(part 1 of 2)
# Autodesk Inventor assembly: Почти готово_CPY
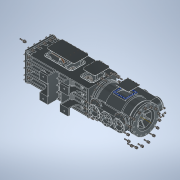
[picture p0: Inventor's stored thumbnail of the model, 180x180]
Saved by Autodesk Inventor 2021 (Build 250183000, 183)
## iProperties
Created: 2020-12-08
Part Number: Почти готово_CPY
Document SubType Name: Assembly
Designer: Тимоха
Author: Тимоха
## Documents named in this file (76)
- C:\Users\Тимоха\Desktop\КР Компрессор\compressor\Почти готово_CPY.iam
- C:\Users\Тимоха\Desktop\КР Компрессор\compressor\Фонарь_CPY.ipt
- C:\Users\Тимоха\Desktop\КР Компрессор\compressor\Башмак_CPY.ipt
- C:\Users\Тимоха\Desktop\КР Компрессор\compressor\Втулка палец шатун_CPY.ipt
- C:\Users\Тимоха\Desktop\КР Компрессор\compressor\Втулка под палец_CPY.ipt
- C:\Users\Тимоха\Desktop\КР Компрессор\compressor\Гайка шток_CPY.ipt
- C:\Users\Тимоха\Desktop\КР Компрессор\compressor\Крейцкопф_CPY.ipt
- C:\Users\Тимоха\Desktop\КР Компрессор\compressor\Палец_CPY.ipt
- C:\Users\Тимоха\Desktop\КР Компрессор\compressor\Стопорное кольцо_CPY.ipt
- C:\Users\Тимоха\Desktop\КР Компрессор\compressor\Верхняя часть поршня_CPY.ipt
- C:\Users\Тимоха\Desktop\КР Компрессор\compressor\Втулка_CPY.ipt
- C:\Users\Тимоха\Desktop\КР Компрессор\compressor\Гайка шток-поршень_CPY.ipt
- C:\Users\Тимоха\Desktop\КР Компрессор\compressor\Кольцо поршень-шток верх_CPY.ipt
- C:\Users\Тимоха\Desktop\КР Компрессор\compressor\Кольцо поршень-шток низ_CPY.ipt
- C:\Users\Тимоха\Desktop\КР Компрессор\compressor\Кольцо поршня_CPY.ipt
- C:\Users\Тимоха\Desktop\КР Компрессор\compressor\Кольцо сальника_CPY.ipt
- C:\Users\Тимоха\Desktop\КР Компрессор\compressor\Корпус дросселя_CPY.ipt
- C:\Users\Тимоха\Desktop\КР Компрессор\compressor\Корпус сальника_CPY.ipt
- C:\Users\Тимоха\Desktop\КР Компрессор\compressor\Крышка стакана_CPY.ipt
- C:\Users\Тимоха\Desktop\КР Компрессор\compressor\Крышка цилиндра 1_CPY.ipt
- C:\Users\Тимоха\Desktop\КР Компрессор\compressor\Крышка цилиндра 2_CPY.ipt
- C:\Users\Тимоха\Desktop\КР Компрессор\compressor\Нижняя часть поршня_CPY.ipt
- C:\Users\Тимоха\Desktop\КР Компрессор\compressor\Опорное кольцо_CPY.ipt
- C:\Users\Тимоха\Desktop\КР Компрессор\compressor\Пружина дросселя_CPY.ipt
- C:\Users\Тимоха\Desktop\КР Компрессор\compressor\Пружина сальника_CPY.ipt
- C:\Users\Тимоха\Desktop\КР Компрессор\compressor\Цилиндр2_CPY.ipt
- C:\Users\Тимоха\Desktop\КР Компрессор\compressor\Клапан1_CPY.iam
- C:\Users\Тимоха\Desktop\КР Компрессор\compressor\Прокладка клапана_CPY.ipt
- C:\Users\Тимоха\Desktop\КР Компрессор\compressor\Стакан1_CPY.ipt
- C:\Users\Тимоха\Desktop\КР Компрессор\compressor\Дроссельное кольцо_CPY.ipt
- C:\Users\Тимоха\Desktop\КР Компрессор\compressor\Уплотнительное кольцо_CPY.ipt
- C:\Users\Тимоха\Desktop\КР Компрессор\compressor\Уплотнение фонарь_CPY.ipt
- C:\Users\Тимоха\Desktop\КР Компрессор\compressor\Крышка сальников_CPY.ipt
- C:\Users\Тимоха\Desktop\КР Компрессор\compressor\Корпус маслосъемника_CPY.ipt
- C:\Users\Тимоха\Desktop\КР Компрессор\compressor\Корпус сальника перегородка 1_CPY.ipt
- C:\Users\Тимоха\Desktop\КР Компрессор\compressor\Крышка перегородки11_CPY.ipt
- C:\Users\Тимоха\Desktop\КР Компрессор\compressor\Крышка перегородки12_CPY.ipt
- C:\Users\Тимоха\Desktop\КР Компрессор\compressor\Крышка перегородки21_CPY.ipt
- C:\Users\Тимоха\Desktop\КР Компрессор\compressor\Крышка перегородки22_CPY.ipt
- C:\Users\Тимоха\Desktop\КР Компрессор\compressor\Маслосъемная пружина_CPY.ipt
- C:\Users\Тимоха\Desktop\КР Компрессор\compressor\Маслосъемное кольцо_CPY.ipt
- C:\Users\Тимоха\Desktop\КР Компрессор\compressor\Придав перегородки1_CPY.ipt
- C:\Users\Тимоха\Desktop\КР Компрессор\compressor\Фланецгайка_CPY.ipt
- C:\Users\Тимоха\Desktop\КР Компрессор\compressor\Шток_CPY.ipt
- C:\Users\Тимоха\Desktop\КР Компрессор\compressor\Прокладка крейцкопф_CPY.ipt
- C:\Users\Тимоха\Documents\Inventor\Content Center Files\R2021\ru-RU\Stud GOST 22038-76\Шпилька M24-6g×70 ГОСТ 22038-76.ipt
- C:\Users\Тимоха\Documents\Inventor\Content Center Files\R2021\ru-RU\Nut GOST 15524-70\Гайка M24-6H ГОСТ 15524-70.ipt
- C:\Users\Тимоха\Documents\Inventor\Content Center Files\R2021\ru-RU\GOST 11371-78  A\Шайба 24 ГОСТ 11371-78.ipt
- C:\Users\Тимоха\Documents\Inventor\Content Center Files\R2021\ru-RU\GOST 15521-70\Гайка M20-6H ГОСТ 15521-70.ipt
- C:\Users\Тимоха\Documents\Inventor\Content Center Files\R2021\ru-RU\Stud GOST 22034-76\Шпилька M20-6g×50 ГОСТ 22034-76.ipt
- C:\Users\Тимоха\Documents\Inventor\Content Center Files\R2021\ru-RU\GOST 10450-78\Шайба 19 ГОСТ 10450-78.ipt
- C:\Users\Тимоха\Documents\Inventor\Content Center Files\R2021\ru-RU\Stud GOST 22038-76\Шпилька M20-6g×85 ГОСТ 22038-76.ipt
- C:\Users\Тимоха\Documents\Inventor\Content Center Files\R2021\ru-RU\GOST 10450-78\Шайба 21 ГОСТ 10450-78.ipt
- C:\Users\Тимоха\Documents\Inventor\Content Center Files\R2021\ru-RU\Nut GOST 15524-70\Гайка M20-6H ГОСТ 15524-70.ipt
- C:\Users\Тимоха\Documents\Inventor\Content Center Files\R2021\ru-RU\GOST 11738-84\Винт M10-6gx35 ГОСТ 11738-84.ipt
- C:\Users\Тимоха\Documents\Inventor\Content Center Files\R2021\ru-RU\GOST 11371-78  A\Шайба 12 ГОСТ 11371-78.ipt
- C:\Users\Тимоха\Documents\Inventor\Content Center Files\R2021\ru-RU\GOST 11738-84\Винт M10-6gx30 ГОСТ 11738-84.ipt
- C:\Users\Тимоха\Documents\Inventor\Content Center Files\R2021\ru-RU\GOST 11738-84\Винт M10-6gx25 ГОСТ 11738-84.ipt
- C:\Users\Тимоха\Documents\Inventor\Content Center Files\R2021\ru-RU\Stud GOST 22038-76\Шпилька M24-6g×80 ГОСТ 22038-76.ipt
- C:\Users\Тимоха\Documents\Inventor\Content Center Files\R2021\ru-RU\GOST 11371-78  A\Шайба 27 ГОСТ 11371-78.ipt
- C:\Users\Тимоха\Desktop\КР Компрессор\compressor\Крышка стакана_MIR_CPY.ipt
- C:\Users\Тимоха\Desktop\КР Компрессор\compressor\Деталь5_CPY.ipt
- C:\Users\Тимоха\Desktop\КР Компрессор\compressor\Деталь6_CPY.ipt
- C:\Users\Тимоха\Documents\Inventor\Content Center Files\R2021\ru-RU\GOST 11371-78  A\Шайба 22 ГОСТ 11371-78.ipt
- C:\Users\Тимоха\Documents\Inventor\Content Center Files\R2021\ru-RU\Bolt GOST R 50274-92\Болт M8-6g×16-F ГОСТ Р 50274-92.ipt
- C:\Users\Тимоха\Desktop\КР Компрессор\compressor\Прокладка крышки фонаря 1_CPY.ipt
- C:\Users\Тимоха\Desktop\КР Компрессор\compressor\Прокладка крышки фонаря 2_CPY.ipt
- C:\Users\Тимоха\Desktop\КР Компрессор\compressor\Маслоотражательное кольцо_CPY.ipt
- C:\Users\Тимоха\Desktop\КР Компрессор\compressor\Прокладка крышки фонаря 1_CPY_MIR.ipt
- C:\Users\Тимоха\Desktop\КР Компрессор\compressor\Прокладка крышки фонаря 2_CPY_MIR.ipt
- C:\Users\Тимоха\Desktop\КР Компрессор\compressor\Крышка фонаря 1.ipt
- C:\Users\Тимоха\Desktop\КР Компрессор\compressor\Крышка фонаря 2.ipt
- C:\Users\Тимоха\Desktop\КР Компрессор\compressor\Крышка фонаря 1_MIR1.ipt
- C:\Users\Тимоха\Desktop\КР Компрессор\compressor\Крышка фонаря 2_MIR1.ipt
- C:\Users\Тимоха\Desktop\КР Компрессор\compressor\Деталь6_CPY_MIR.ipt
- C:\Users\Тимоха\Desktop\КР Компрессор\compressor\Деталь5_CPY_MIR.ipt
## Components (627 placed, 75 different names)
1. Фонарь_CPY:1 — Заподлицо:5, Заподлицо:4, Заподлицо:7, Заподлицо:6, Цилиндрический:2, Жесткий:70, Жесткий:69, Жесткий:94, Жесткий:98, Жесткий:97, Жесткий:106, Жесткий:127, Жесткий:163, Жесткий:165, Жесткий:166, Жесткий:164, Жесткий:171, Жесткий:173, Жесткий:174, Жесткий:172, Жесткий:169, Жесткий:167, Жесткий:170, Жесткий:168, Жесткий:192, Жесткий:197, Жесткий:191, Жесткий:196, Жесткий:194, Жесткий:193, Жесткий:195, Заподлицо:9, Заподлицо:10, Заподлицо:11, Заподлицо:12
2. Башмак_CPY:1 — Цилиндрический:2, Жесткий:4
3. Втулка палец шатун_CPY:1 — Жесткий:3
4. Втулка под палец_CPY:1 — Жесткий:1, С поворотом:1
5. Гайка шток_CPY:1 — Жесткий:110
6. Крейцкопф_CPY:1 — Жесткий:4, Жесткий:1, Жесткий:2, Жесткий:5, Жесткий:206, Жесткий:208, Жесткий:209
7. Втулка под палец_CPY:2 — Жесткий:3, Жесткий:2
8. Башмак_CPY:2 — Жесткий:5
9. Палец_CPY:1 — С поворотом:1, Жесткий:7, Жесткий:6
10. Стопорное кольцо_CPY:1 — Жесткий:7
11. Стопорное кольцо_CPY:2 — Жесткий:6
12. Верхняя часть поршня_CPY:1 — Совмещение:1, Жесткий:13, Жесткий:9, Жесткий:8, Жесткий:20
13. Втулка_CPY:1 — Жесткий:16, Жесткий:15, Цилиндрический:1
14. Гайка шток-поршень_CPY:1 — Жесткий:14, Жесткий:107
15. Кольцо поршень-шток верх_CPY:1 — Жесткий:14, Жесткий:13
16. Кольцо поршень-шток низ_CPY:1 — Жесткий:12
17. Кольцо поршня_CPY:1 — Жесткий:9
18. Кольцо сальника_CPY:1 — Жесткий:27, Жесткий:31, Жесткий:30
19. Корпус дросселя_CPY:1 — С поворотом:3, Жесткий:26, Жесткий:62
20. Корпус сальника_CPY:1 — С поворотом:3, Жесткий:32, Жесткий:57
21. Крышка стакана_CPY:1 — Жесткий:23
22. Крышка цилиндра 1_CPY:1 — Совмещение:1, Жесткий:16, Жесткий:112
23. Крышка цилиндра 2_CPY:1 — Жесткий:70, Жесткий:79, Жесткий:61, Жесткий:78, Жесткий:125
24. Нижняя часть поршня_CPY:1 — Жесткий:12, Жесткий:8, Жесткий:21, Жесткий:11, Жесткий:10
25. Опорное кольцо_CPY:1 — Жесткий:21
26. Пружина дросселя_CPY:1 — Жесткий:25
27. Пружина сальника_CPY:1 — Жесткий:27
28. Цилиндр2_CPY:1 — Заподлицо:2, Жесткий:79, Жесткий:23, Жесткий:15, Жесткий:80, Жесткий:18, Жесткий:81, Жесткий:111, Жесткий:116, Жесткий:115, Жесткий:117, Жесткий:118, Жесткий:119, Жесткий:122, Жесткий:461
29. Кольцо поршня_CPY:2 — Жесткий:11
30. Кольцо поршня_CPY:3 — Цилиндрический:1, Жесткий:10
31. Клапан1_CPY:1 [sub-assembly] — Жесткий:80
32. Прокладка клапана_CPY:1 — Жесткий:18
33. Стакан1_CPY:1 — Жесткий:81
34. Опорное кольцо_CPY:2 — Жесткий:20
35. Дроссельное кольцо_CPY:1 — Жесткий:26, Жесткий:25
36. Кольцо сальника_CPY:2 — Жесткий:32, Жесткий:31, Жесткий:28
37. Пружина сальника_CPY:2 — Жесткий:28
38. Кольцо сальника_CPY:3 — Жесткий:30, Жесткий:29
39. Пружина сальника_CPY:3 — Жесткий:29
40. Кольцо сальника_CPY:4 — Жесткий:33, Жесткий:37, Жесткий:36
41. Корпус сальника_CPY:2 — Жесткий:57, Жесткий:38, Жесткий:58
42. Пружина сальника_CPY:4 — Жесткий:33
43. Кольцо сальника_CPY:5 — Жесткий:38, Жесткий:37, Жесткий:34
44. Пружина сальника_CPY:5 — Жесткий:34
45. Кольцо сальника_CPY:6 — Жесткий:36, Жесткий:35
46. Пружина сальника_CPY:6 — Жесткий:35
47. Кольцо сальника_CPY:7 — Жесткий:39, Жесткий:43, Жесткий:42
48. Корпус сальника_CPY:3 — Жесткий:58, Жесткий:44, Жесткий:59
49. Пружина сальника_CPY:7 — Жесткий:39
50. Кольцо сальника_CPY:8 — Жесткий:44, Жесткий:43, Жесткий:40
51. Пружина сальника_CPY:8 — Жесткий:40
52. Кольцо сальника_CPY:9 — Жесткий:42, Жесткий:41
53. Пружина сальника_CPY:9 — Жесткий:41
54. Кольцо сальника_CPY:10 — Жесткий:45, Жесткий:49, Жесткий:48
55. Корпус сальника_CPY:4 — Жесткий:59, Жесткий:50, Жесткий:60
56. Пружина сальника_CPY:10 — Жесткий:45
57. Кольцо сальника_CPY:11 — Жесткий:50, Жесткий:49, Жесткий:46
58. Пружина сальника_CPY:11 — Жесткий:46
59. Кольцо сальника_CPY:12 — Жесткий:48, Жесткий:47
60. Пружина сальника_CPY:12 — Жесткий:47
61. Кольцо сальника_CPY:13 — Жесткий:51, Жесткий:55, Жесткий:54
62. Корпус сальника_CPY:5 — Жесткий:60, Жесткий:56, Жесткий:77
63. Пружина сальника_CPY:13 — Жесткий:51
64. Кольцо сальника_CPY:14 — Жесткий:56, Жесткий:55, Жесткий:52
65. Пружина сальника_CPY:14 — Жесткий:52
66. Кольцо сальника_CPY:15 — Жесткий:54, Жесткий:53
67. Пружина сальника_CPY:15 — Жесткий:53
68. Уплотнительное кольцо_CPY:1 — Жесткий:62, Жесткий:61
69. Кольцо сальника_CPY:16 — Жесткий:63, Жесткий:67, Жесткий:66
70. Пружина сальника_CPY:16 — Жесткий:63
71. Кольцо сальника_CPY:17 — Жесткий:67, Жесткий:64, Жесткий:103
72. Пружина сальника_CPY:17 — Жесткий:64
73. Кольцо сальника_CPY:18 — Жесткий:66, Жесткий:65
74. Пружина сальника_CPY:18 — Жесткий:65
75. Уплотнение фонарь_CPY:1 — Жесткий:69
76. Кольцо сальника_CPY:19 — Жесткий:71, Жесткий:75, Жесткий:74
77. Корпус сальника_CPY:6 — Жесткий:77, Жесткий:76
78. Пружина сальника_CPY:19 — Жесткий:71
79. Кольцо сальника_CPY:20 — Жесткий:76, Жесткий:75, Жесткий:72
80. Пружина сальника_CPY:20 — Жесткий:72
81. Кольцо сальника_CPY:21 — Жесткий:74, Жесткий:73
82. Пружина сальника_CPY:21 — Жесткий:73
83. Крышка сальников_CPY:1 — Жесткий:78
84. Корпус маслосъемника_CPY:1 — Жесткий:104, Жесткий:102
85. Корпус сальника перегородка 1_CPY:1 — Жесткий:95, Жесткий:96, Жесткий:87, Жесткий:93
86. Крышка перегородки11_CPY:1 — Жесткий:95, Жесткий:94
87. Крышка перегородки12_CPY:1 — Жесткий:96, Жесткий:128
88. Крышка перегородки21_CPY:1 — Жесткий:104, Жесткий:103, Жесткий:98, Жесткий:105
89. Крышка перегородки22_CPY:1 — Жесткий:105, Жесткий:130
90. Маслосъемная пружина_CPY:1 — Жесткий:99
91. Маслосъемное кольцо_CPY:1 — Жесткий:99, Жесткий:101
92. Придав перегородки1_CPY:1 — Жесткий:97, Жесткий:134
93. Кольцо сальника_CPY:22 — Жесткий:82, Жесткий:86, Жесткий:85
94. Пружина сальника_CPY:22 — Жесткий:82
95. Кольцо сальника_CPY:23 — Жесткий:87, Жесткий:86, Жесткий:83
96. Пружина сальника_CPY:23 — Жесткий:83
97. Кольцо сальника_CPY:24 — Жесткий:85, Жесткий:84
98. Пружина сальника_CPY:24 — Жесткий:84
99. Кольцо сальника_CPY:25 — Жесткий:88, Жесткий:92, Жесткий:91
100. Пружина сальника_CPY:25 — Жесткий:88
101. Кольцо сальника_CPY:26 — Жесткий:93, Жесткий:92, Жесткий:89
102. Пружина сальника_CPY:26 — Жесткий:89
103. Кольцо сальника_CPY:27 — Жесткий:91, Жесткий:90
104. Пружина сальника_CPY:27 — Жесткий:90
105. Маслосъемная пружина_CPY:2 — Жесткий:100
106. Маслосъемное кольцо_CPY:2 — Жесткий:102, Жесткий:101, Жесткий:100
107. Придав перегородки1_CPY:2 — Жесткий:106, Жесткий:132
108. Фланецгайка_CPY:1 — Жесткий:207
109. Шток_CPY:1 — Жесткий:110, Жесткий:107, Жесткий:404
110. Прокладка крейцкопф_CPY:1 — Жесткий:207, Жесткий:206
111. Шпилька ГОСТ 22038-76 M24-6g×70:2 — Жесткий:114
112. Гайка ГОСТ 15524-70 M24:2 — Жесткий:114
113. Шайба  ГОСТ 11371-78 25:2 — Совмещение:2
114. Шпилька ГОСТ 22038-76 M24-6g×70:3
115. Гайка ГОСТ 15524-70 M24:3
116. Шайба  ГОСТ 11371-78 25:3
117. Шпилька ГОСТ 22038-76 M24-6g×70:4
118. Гайка ГОСТ 15524-70 M24:4
119. Шайба  ГОСТ 11371-78 25:4
120. Шпилька ГОСТ 22038-76 M24-6g×70:5
121. Гайка ГОСТ 15524-70 M24:5
122. Шайба  ГОСТ 11371-78 25:5
123. Шпилька ГОСТ 22038-76 M24-6g×70:6
124. Гайка ГОСТ 15524-70 M24:6
125. Шайба  ГОСТ 11371-78 25:6
126. Шпилька ГОСТ 22038-76 M24-6g×70:7
127. Гайка ГОСТ 15524-70 M24:7
128. Шайба  ГОСТ 11371-78 25:7
129. Шпилька ГОСТ 22038-76 M24-6g×70:8
130. Гайка ГОСТ 15524-70 M24:8
131. Шайба  ГОСТ 11371-78 25:8
132. Шпилька ГОСТ 22038-76 M24-6g×70:9
133. Гайка ГОСТ 15524-70 M24:9
134. Шайба  ГОСТ 11371-78 25:9
135. Шпилька ГОСТ 22038-76 M24-6g×70:10
136. Гайка ГОСТ 15524-70 M24:10
137. Шайба  ГОСТ 11371-78 25:10
138. Шпилька ГОСТ 22038-76 M24-6g×70:11
139. Гайка ГОСТ 15524-70 M24:11
140. Шайба  ГОСТ 11371-78 25:11
141. Шпилька ГОСТ 22038-76 M24-6g×70:12
142. Гайка ГОСТ 15524-70 M24:12
143. Шайба  ГОСТ 11371-78 25:12
144. Шпилька ГОСТ 22038-76 M24-6g×70:13
145. Гайка ГОСТ 15524-70 M24:13
146. Шайба  ГОСТ 11371-78 25:13
147. Шпилька ГОСТ 22038-76 M24-6g×70:14
148. Гайка ГОСТ 15524-70 M24:14
149. Шайба  ГОСТ 11371-78 25:14
150. Шпилька ГОСТ 22038-76 M24-6g×70:15
151. Гайка ГОСТ 15524-70 M24:15
152. Шайба  ГОСТ 11371-78 25:15
153. Шпилька ГОСТ 22038-76 M24-6g×70:16
154. Гайка ГОСТ 15524-70 M24:16
155. Шайба  ГОСТ 11371-78 25:16
156. Шпилька ГОСТ 22038-76 M24-6g×70:17
157. Гайка ГОСТ 15524-70 M24:17
158. Шайба  ГОСТ 11371-78 25:17
159. Клапан1_CPY:2 [sub-assembly] — Жесткий:116
160. Прокладка клапана_CPY:2 — Жесткий:115
161. Стакан1_CPY:2 — Жесткий:117
162. Крышка стакана_CPY:2 — Жесткий:118
163. Шпилька ГОСТ 22038-76 M24-6g×80:1 — Жесткий:138, Жесткий:137
164. Гайка ГОСТ 15524-70 M24:18 — Жесткий:138
165. Шайба  ГОСТ 11371-78 28:1 — Жесткий:137
166. Шпилька ГОСТ 22038-76 M24-6g×80:2 — Жесткий:140, Жесткий:139
167. Гайка ГОСТ 15524-70 M24:19 — Жесткий:140
168. Шайба  ГОСТ 11371-78 28:2 — Жесткий:163, Жесткий:139
169. Шпилька ГОСТ 22038-76 M24-6g×80:3 — Жесткий:142, Жесткий:141
170. Гайка ГОСТ 15524-70 M24:20 — Жесткий:142
171. Шайба  ГОСТ 11371-78 28:3 — Жесткий:165, Жесткий:141
172. Шпилька ГОСТ 22038-76 M24-6g×80:4 — Жесткий:144, Жесткий:143
173. Гайка ГОСТ 15524-70 M24:21 — Жесткий:144
174. Шайба  ГОСТ 11371-78 28:4 — Жесткий:166, Жесткий:143
175. Шпилька ГОСТ 22038-76 M24-6g×80:5 — Жесткий:146, Жесткий:145
176. Гайка ГОСТ 15524-70 M24:22 — Жесткий:146
177. Шайба  ГОСТ 11371-78 28:5 — Жесткий:164, Жесткий:145
178. Шпилька ГОСТ 22038-76 M24-6g×80:6 — Жесткий:148, Жесткий:147
179. Гайка ГОСТ 15524-70 M24:23 — Жесткий:148
180. Шайба  ГОСТ 11371-78 28:6 — Жесткий:171, Жесткий:147
181. Шпилька ГОСТ 22038-76 M24-6g×80:7 — Жесткий:150, Жесткий:149
182. Гайка ГОСТ 15524-70 M24:24 — Жесткий:150
183. Шайба  ГОСТ 11371-78 28:7 — Жесткий:173, Жесткий:149
184. Шпилька ГОСТ 22038-76 M24-6g×80:8 — Жесткий:152, Жесткий:151
185. Гайка ГОСТ 15524-70 M24:25 — Жесткий:152
186. Шайба  ГОСТ 11371-78 28:8 — Жесткий:174, Жесткий:151
187. Шпилька ГОСТ 22038-76 M24-6g×80:9 — Жесткий:154, Жесткий:153
188. Гайка ГОСТ 15524-70 M24:26 — Жесткий:154
189. Шайба  ГОСТ 11371-78 28:9 — Жесткий:172, Жесткий:153
190. Шпилька ГОСТ 22038-76 M24-6g×80:10 — Жесткий:156, Жесткий:155
191. Гайка ГОСТ 15524-70 M24:27 — Жесткий:156
192. Шайба  ГОСТ 11371-78 28:10 — Жесткий:169, Жесткий:155
193. Шпилька ГОСТ 22038-76 M24-6g×80:11 — Жесткий:158, Жесткий:157
194. Гайка ГОСТ 15524-70 M24:28 — Жесткий:158
195. Шайба  ГОСТ 11371-78 28:11 — Жесткий:167, Жесткий:157
196. Шпилька ГОСТ 22038-76 M24-6g×80:12 — Жесткий:160, Жесткий:159
197. Гайка ГОСТ 15524-70 M24:29 — Жесткий:160
198. Шайба  ГОСТ 11371-78 28:12 — Жесткий:170, Жесткий:159
199. Шпилька ГОСТ 22038-76 M24-6g×80:13 — Жесткий:162, Жесткий:161
200. Гайка ГОСТ 15524-70 M24:30 — Жесткий:162
201. Шайба  ГОСТ 11371-78 28:13 — Жесткий:168, Жесткий:161
202. Шпилька ГОСТ 22038-76 M24-6g×80:14 — Жесткий:176, Жесткий:175
203. Гайка ГОСТ 15524-70 M24:31 — Жесткий:176
204. Шайба  ГОСТ 11371-78 28:14 — Жесткий:192, Жесткий:175
205. Шпилька ГОСТ 22038-76 M24-6g×80:15 — Жесткий:178, Жесткий:177
206. Гайка ГОСТ 15524-70 M24:32 — Жесткий:178
207. Шайба  ГОСТ 11371-78 28:15 — Жесткий:197, Жесткий:177
208. Шпилька ГОСТ 22038-76 M24-6g×80:16 — Жесткий:180, Жесткий:179
209. Гайка ГОСТ 15524-70 M24:33 — Жесткий:180
210. Шайба  ГОСТ 11371-78 28:16 — Жесткий:191, Жесткий:179
211. Шпилька ГОСТ 22038-76 M24-6g×80:17 — Жесткий:184, Жесткий:183
212. Гайка ГОСТ 15524-70 M24:34 — Жесткий:184
213. Шайба  ГОСТ 11371-78 28:17 — Жесткий:196, Жесткий:183
214. Шпилька ГОСТ 22038-76 M24-6g×80:18 — Жесткий:186, Жесткий:185
215. Гайка ГОСТ 15524-70 M24:35 — Жесткий:186
216. Шайба  ГОСТ 11371-78 28:18 — Жесткий:194, Жесткий:185
217. Шпилька ГОСТ 22038-76 M24-6g×80:19 — Жесткий:188, Жесткий:187
218. Гайка ГОСТ 15524-70 M24:36 — Жесткий:188
219. Шайба  ГОСТ 11371-78 28:19 — Жесткий:193, Жесткий:187
220. Шпилька ГОСТ 22038-76 M24-6g×80:20 — Жесткий:190, Жесткий:189
221. Гайка ГОСТ 15524-70 M24:37 — Жесткий:190
222. Шайба  ГОСТ 11371-78 28:20 — Жесткий:195, Жесткий:189
223. Крышка стакана_MIR_CPY:1
224. Крышка стакана_MIR_CPY:2
225. Деталь6_CPY:2
226. Шпилька ГОСТ 22038-76 M20-6g×85:2 — Жесткий:208, Жесткий:211, Жесткий:210
227. Шпилька ГОСТ 22038-76 M20-6g×85:3 — Жесткий:209, Жесткий:213, Жесткий:212
228. Гайка ГОСТ 15524-70 M20:2 — Жесткий:211
229. Шайба  ГОСТ 11371-78 23:1 — Жесткий:210
230. Гайка ГОСТ 15524-70 M20:3 — Жесткий:213
231. Шайба  ГОСТ 11371-78 23:2 — Жесткий:212
232. Прокладка крышки фонаря 1_CPY:1 — Заподлицо:5, Заподлицо:4
233. Прокладка крышки фонаря 2_CPY:1 — Заподлицо:7, Заподлицо:6
234. Маслоотражательное кольцо_CPY:1 — Жесткий:404
235. Прокладка крышки фонаря 1_CPY_MIR:1
236. Прокладка крышки фонаря 2_CPY_MIR:1
237. Крышка фонаря 1:1 — Заподлицо:9, Заподлицо:10, Жесткий:395, Жесткий:396, Жесткий:397, Жесткий:398, Жесткий:399, Жесткий:400, Жесткий:401, Жесткий:402, Жесткий:403, Жесткий:404, Жесткий:405, Жесткий:406
238. Крышка фонаря 2:1 — Заподлицо:11, Заподлицо:12, С поворотом:3, С поворотом:4, С поворотом:5, Жесткий:407, Жесткий:408, Жесткий:409, Жесткий:410, Жесткий:411, Жесткий:412, Жесткий:413, Жесткий:414, Жесткий:415, Жесткий:416, Жесткий:417, Жесткий:418, Жесткий:419, Жесткий:420, Жесткий:421, Жесткий:422, Жесткий:423, Жесткий:424, Жесткий:425, Жесткий:426, Жесткий:427
239. Болт ГОСТ Р 50274-92 M8-6g×16-F:65 — Жесткий:400
240. Болт ГОСТ Р 50274-92 M8-6g×16-F:66 — Жесткий:424
241. Болт ГОСТ Р 50274-92 M8-6g×16-F:69 — С поворотом:3
242. Болт ГОСТ Р 50274-92 M8-6g×16-F:70 — С поворотом:4
243. Болт ГОСТ Р 50274-92 M8-6g×16-F:71 — Жесткий:410
244. Болт ГОСТ Р 50274-92 M8-6g×16-F:72 — Жесткий:416
245. Болт ГОСТ Р 50274-92 M8-6g×16-F:74 — Жесткий:415
246. Болт ГОСТ Р 50274-92 M8-6g×16-F:76 — Жесткий:419
247. Болт ГОСТ Р 50274-92 M8-6g×16-F:77 — Жесткий:414
248. Болт ГОСТ Р 50274-92 M8-6g×16-F:78 — Жесткий:417
249. Болт ГОСТ Р 50274-92 M8-6g×16-F:79 — Жесткий:421
250. Болт ГОСТ Р 50274-92 M8-6g×16-F:80 — Жесткий:427
251. Болт ГОСТ Р 50274-92 M8-6g×16-F:82 — Жесткий:422
252. Болт ГОСТ Р 50274-92 M8-6g×16-F:83 — С поворотом:5
253. Болт ГОСТ Р 50274-92 M8-6g×16-F:87 — Жесткий:409
254. Болт ГОСТ Р 50274-92 M8-6g×16-F:88 — Жесткий:420
255. Болт ГОСТ Р 50274-92 M8-6g×16-F:89 — Жесткий:423
256. Болт ГОСТ Р 50274-92 M8-6g×16-F:92 — Жесткий:408
257. Болт ГОСТ Р 50274-92 M8-6g×16-F:95 — Жесткий:407
258. Болт ГОСТ Р 50274-92 M8-6g×16-F:96 — Жесткий:425
259. Болт ГОСТ Р 50274-92 M8-6g×16-F:101 — Жесткий:395
260. Болт ГОСТ Р 50274-92 M8-6g×16-F:102 — Жесткий:406
261. Болт ГОСТ Р 50274-92 M8-6g×16-F:104 — Жесткий:397
262. Болт ГОСТ Р 50274-92 M8-6g×16-F:105 — Жесткий:396
263. Болт ГОСТ Р 50274-92 M8-6g×16-F:106 — Жесткий:398
264. Болт ГОСТ Р 50274-92 M8-6g×16-F:107 — Жесткий:402
265. Болт ГОСТ Р 50274-92 M8-6g×16-F:108 — Жесткий:404
266. Болт ГОСТ Р 50274-92 M8-6g×16-F:110 — Жесткий:403
267. Болт ГОСТ Р 50274-92 M8-6g×16-F:114 — Жесткий:405
268. Болт ГОСТ Р 50274-92 M8-6g×16-F:115 — Жесткий:411
269. Болт ГОСТ Р 50274-92 M8-6g×16-F:118 — Жесткий:426
270. Болт ГОСТ Р 50274-92 M8-6g×16-F:119 — Жесткий:399
271. Болт ГОСТ Р 50274-92 M8-6g×16-F:123 — Жесткий:401
272. Болт ГОСТ Р 50274-92 M8-6g×16-F:124 — Жесткий:412
273. Болт ГОСТ Р 50274-92 M8-6g×16-F:128 — Жесткий:413
274. Болт ГОСТ Р 50274-92 M8-6g×16-F:132 — Жесткий:418
275. Крышка фонаря 1_MIR1:1 — Жесткий:428, Жесткий:445, Жесткий:446, Жесткий:447, Жесткий:448, Жесткий:449, Жесткий:450, Жесткий:451, Жесткий:452, Жесткий:453, Жесткий:456, Жесткий:457
276. Крышка фонаря 2_MIR1:1 — Жесткий:429, С поворотом:6, С поворотом:7, Жесткий:430, Жесткий:431, Жесткий:432, Жесткий:433, Жесткий:434, Жесткий:435, Жесткий:436, Жесткий:437, Жесткий:438, С поворотом:8, Жесткий:439, Жесткий:440, Жесткий:441, Жесткий:442, Жесткий:443, Жесткий:444, Жесткий:454, Жесткий:455, Жесткий:458, Жесткий:459, Жесткий:460
277. Болт ГОСТ Р 50274-92 M8-6g×16-F:133 — Жесткий:428
278. Болт ГОСТ Р 50274-92 M8-6g×16-F:134 — Жесткий:429
279. Болт ГОСТ Р 50274-92 M8-6g×16-F:135 — С поворотом:6
280. Болт ГОСТ Р 50274-92 M8-6g×16-F:136 — С поворотом:7
281. Болт ГОСТ Р 50274-92 M8-6g×16-F:137 — Жесткий:430
282. Болт ГОСТ Р 50274-92 M8-6g×16-F:138 — Жесткий:431
283. Болт ГОСТ Р 50274-92 M8-6g×16-F:139 — Жесткий:432
284. Болт ГОСТ Р 50274-92 M8-6g×16-F:140 — Жесткий:433
285. Болт ГОСТ Р 50274-92 M8-6g×16-F:141 — Жесткий:434
286. Болт ГОСТ Р 50274-92 M8-6g×16-F:142 — Жесткий:435
287. Болт ГОСТ Р 50274-92 M8-6g×16-F:143 — Жесткий:436
288. Болт ГОСТ Р 50274-92 M8-6g×16-F:144 — Жесткий:437
289. Болт ГОСТ Р 50274-92 M8-6g×16-F:145 — Жесткий:438
290. Болт ГОСТ Р 50274-92 M8-6g×16-F:146 — С поворотом:8
291. Болт ГОСТ Р 50274-92 M8-6g×16-F:147 — Жесткий:439
292. Болт ГОСТ Р 50274-92 M8-6g×16-F:148 — Жесткий:440
293. Болт ГОСТ Р 50274-92 M8-6g×16-F:149 — Жесткий:441
294. Болт ГОСТ Р 50274-92 M8-6g×16-F:150 — Жесткий:442
295. Болт ГОСТ Р 50274-92 M8-6g×16-F:151 — Жесткий:443
296. Болт ГОСТ Р 50274-92 M8-6g×16-F:152 — Жесткий:444
297. Болт ГОСТ Р 50274-92 M8-6g×16-F:153 — Жесткий:445
298. Болт ГОСТ Р 50274-92 M8-6g×16-F:154 — Жесткий:446
299. Болт ГОСТ Р 50274-92 M8-6g×16-F:155 — Жесткий:447
300. Болт ГОСТ Р 50274-92 M8-6g×16-F:156 — Жесткий:448
301. Болт ГОСТ Р 50274-92 M8-6g×16-F:157 — Жесткий:449
302. Болт ГОСТ Р 50274-92 M8-6g×16-F:158 — Жесткий:450
303. Болт ГОСТ Р 50274-92 M8-6g×16-F:159 — Жесткий:451
304. Болт ГОСТ Р 50274-92 M8-6g×16-F:160 — Жесткий:452
305. Болт ГОСТ Р 50274-92 M8-6g×16-F:161 — Жесткий:453
306. Болт ГОСТ Р 50274-92 M8-6g×16-F:162 — Жесткий:454
307. Болт ГОСТ Р 50274-92 M8-6g×16-F:163 — Жесткий:455
308. Болт ГОСТ Р 50274-92 M8-6g×16-F:164 — Жесткий:456
309. Болт ГОСТ Р 50274-92 M8-6g×16-F:165 — Жесткий:457
310. Болт ГОСТ Р 50274-92 M8-6g×16-F:166 — Жесткий:458
311. Болт ГОСТ Р 50274-92 M8-6g×16-F:167 — Жесткий:459
312. Болт ГОСТ Р 50274-92 M8-6g×16-F:168 — Жесткий:460
313. Болт ГОСТ Р 50274-92 M8-6g×16-F:169 — Жесткий:477
314. Болт ГОСТ Р 50274-92 M8-6g×16-F:170 — Жесткий:475
315. Болт ГОСТ Р 50274-92 M8-6g×16-F:171 — Жесткий:467
316. Болт ГОСТ Р 50274-92 M8-6g×16-F:172 — Жесткий:474
317. Болт ГОСТ Р 50274-92 M8-6g×16-F:173 — Жесткий:473
318. Болт ГОСТ Р 50274-92 M8-6g×16-F:174 — Жесткий:464
319. Болт ГОСТ Р 50274-92 M8-6g×16-F:175 — Жесткий:462
320. Болт ГОСТ Р 50274-92 M8-6g×16-F:178 — Жесткий:466
321. Болт ГОСТ Р 50274-92 M8-6g×16-F:179 — Жесткий:465
322. Болт ГОСТ Р 50274-92 M8-6g×16-F:180 — Жесткий:463
323. Болт ГОСТ Р 50274-92 M8-6g×16-F:187 — Жесткий:476
324. Болт ГОСТ Р 50274-92 M8-6g×16-F:188 — Жесткий:472
325. Болт ГОСТ Р 50274-92 M8-6g×16-F:189 — Жесткий:471
326. Болт ГОСТ Р 50274-92 M8-6g×16-F:190 — Жесткий:470
327. Болт ГОСТ Р 50274-92 M8-6g×16-F:191 — Жесткий:469
328. Болт ГОСТ Р 50274-92 M8-6g×16-F:192 — Жесткий:468
329. Деталь5_CPY:2 — Жесткий:461
330. Деталь6_CPY_MIR:1 — Жесткий:462, Жесткий:463, Жесткий:464, Жесткий:465, Жесткий:466, Жесткий:467, Жесткий:468, Жесткий:469, Жесткий:470, Жесткий:471, Жесткий:472, Жесткий:473, Жесткий:474, Жесткий:475, Жесткий:476, Жесткий:477
331. Болт ГОСТ Р 50274-92 M8-6g×16-F:193
332. Болт ГОСТ Р 50274-92 M8-6g×16-F:194
333. Болт ГОСТ Р 50274-92 M8-6g×16-F:195
334. Болт ГОСТ Р 50274-92 M8-6g×16-F:196
335. Болт ГОСТ Р 50274-92 M8-6g×16-F:197
336. Болт ГОСТ Р 50274-92 M8-6g×16-F:198
337. Болт ГОСТ Р 50274-92 M8-6g×16-F:199
338. Болт ГОСТ Р 50274-92 M8-6g×16-F:200
339. Болт ГОСТ Р 50274-92 M8-6g×16-F:201
340. Болт ГОСТ Р 50274-92 M8-6g×16-F:202
341. Болт ГОСТ Р 50274-92 M8-6g×16-F:203
342. Болт ГОСТ Р 50274-92 M8-6g×16-F:204
343. Болт ГОСТ Р 50274-92 M8-6g×16-F:205
344. Болт ГОСТ Р 50274-92 M8-6g×16-F:206
345. Болт ГОСТ Р 50274-92 M8-6g×16-F:207
346. Болт ГОСТ Р 50274-92 M8-6g×16-F:208
347. Деталь5_CPY_MIR:1
348. Шпилька ГОСТ 22038-76 M20-6g×85:1 — Жесткий:126, Жесткий:125
349. Шайба ГОСТ 10450-78 21:1 — Жесткий:126
350. Гайка ГОСТ 15524-70 M20:1 — Жесткий:127
351. Шпилька ГОСТ 22038-76 M20-6g×85:4
352. Шайба ГОСТ 10450-78 21:2
353. Гайка ГОСТ 15524-70 M20:4
354. Шпилька ГОСТ 22038-76 M20-6g×85:5
355. Шайба ГОСТ 10450-78 21:3
356. Гайка ГОСТ 15524-70 M20:5
357. Шпилька ГОСТ 22038-76 M20-6g×85:6
358. Шайба ГОСТ 10450-78 21:4
359. Гайка ГОСТ 15524-70 M20:6
360. Шпилька ГОСТ 22038-76 M20-6g×85:7
361. Шайба ГОСТ 10450-78 21:5
362. Гайка ГОСТ 15524-70 M20:7
363. Шпилька ГОСТ 22038-76 M20-6g×85:8
364. Шайба ГОСТ 10450-78 21:6
365. Гайка ГОСТ 15524-70 M20:8
366. Шпилька ГОСТ 22038-76 M20-6g×85:9
367. Шайба ГОСТ 10450-78 21:7
368. Гайка ГОСТ 15524-70 M20:9
369. Шпилька ГОСТ 22038-76 M20-6g×85:10
370. Шайба ГОСТ 10450-78 21:8
371. Гайка ГОСТ 15524-70 M20:10
372. Шпилька ГОСТ 22038-76 M20-6g×85:11
373. Шайба ГОСТ 10450-78 21:9
374. Гайка ГОСТ 15524-70 M20:11
375. Шпилька ГОСТ 22038-76 M20-6g×85:12
376. Шайба ГОСТ 10450-78 21:10
377. Гайка ГОСТ 15524-70 M20:12
378. Шпилька ГОСТ 22038-76 M20-6g×85:13
379. Шайба ГОСТ 10450-78 21:11
380. Гайка ГОСТ 15524-70 M20:13
381. Шпилька ГОСТ 22038-76 M20-6g×85:14
382. Шайба ГОСТ 10450-78 21:12
383. Гайка ГОСТ 15524-70 M20:14
384. Шпилька ГОСТ 22038-76 M20-6g×85:15
385. Шайба ГОСТ 10450-78 21:13
386. Гайка ГОСТ 15524-70 M20:15
387. Шпилька ГОСТ 22038-76 M20-6g×85:16
388. Шайба ГОСТ 10450-78 21:14
389. Гайка ГОСТ 15524-70 M20:16
390. Шпилька ГОСТ 22038-76 M20-6g×85:17
391. Шайба ГОСТ 10450-78 21:15
392. Гайка ГОСТ 15524-70 M20:17
393. Шпилька ГОСТ 22038-76 M20-6g×85:18
394. Шайба ГОСТ 10450-78 21:16
395. Гайка ГОСТ 15524-70 M20:18
396. Гайка ГОСТ 15521-70 M20:1 — Жесткий:121
397. Шпилька ГОСТ 22034-76 M20-6g×50:1 — Жесткий:119, Жесткий:121, Жесткий:120
398. Шайба ГОСТ 10450-78 19:1 — Жесткий:120
399. Гайка ГОСТ 15521-70 M20:5
400. Шпилька ГОСТ 22034-76 M20-6g×50:5
401. Шайба ГОСТ 10450-78 19:5
402. Гайка ГОСТ 15521-70 M20:6
403. Шпилька ГОСТ 22034-76 M20-6g×50:6
404. Шайба ГОСТ 10450-78 19:6
405. Гайка ГОСТ 15521-70 M20:7
406. Шпилька ГОСТ 22034-76 M20-6g×50:7
407. Шайба ГОСТ 10450-78 19:7
408. Гайка ГОСТ 15521-70 M20:8
409. Шпилька ГОСТ 22034-76 M20-6g×50:8
410. Шайба ГОСТ 10450-78 19:8
411. Гайка ГОСТ 15521-70 M20:9
412. Шпилька ГОСТ 22034-76 M20-6g×50:9
413. Шайба ГОСТ 10450-78 19:9
414. Гайка ГОСТ 15521-70 M20:10
415. Шпилька ГОСТ 22034-76 M20-6g×50:10
416. Шайба ГОСТ 10450-78 19:10
417. Гайка ГОСТ 15521-70 M20:11
418. Шпилька ГОСТ 22034-76 M20-6g×50:11
419. Шайба ГОСТ 10450-78 19:11
420. Гайка ГОСТ 15521-70 M20:12
421. Шпилька ГОСТ 22034-76 M20-6g×50:12
422. Шайба ГОСТ 10450-78 19:12
423. Гайка ГОСТ 15521-70 M20:13
424. Шпилька ГОСТ 22034-76 M20-6g×50:13
425. Шайба ГОСТ 10450-78 19:13
426. Шпилька ГОСТ 22038-76 M24-6g×70:1 — Жесткий:113, Жесткий:111
427. Гайка ГОСТ 15524-70 M24:1 — Жесткий:113
428. Шайба  ГОСТ 11371-78 25:1 — Заподлицо:1, Жесткий:112
429. Шпилька ГОСТ 22038-76 M24-6g×70:18
430. Гайка ГОСТ 15524-70 M24:38
431. Шайба  ГОСТ 11371-78 25:18
432. Шпилька ГОСТ 22038-76 M24-6g×70:19
433. Гайка ГОСТ 15524-70 M24:39
434. Шайба  ГОСТ 11371-78 25:19
435. Шпилька ГОСТ 22038-76 M24-6g×70:20
436. Гайка ГОСТ 15524-70 M24:40
437. Шайба  ГОСТ 11371-78 25:20
438. Шпилька ГОСТ 22038-76 M24-6g×70:21
439. Гайка ГОСТ 15524-70 M24:41
440. Шайба  ГОСТ 11371-78 25:21
441. Шпилька ГОСТ 22038-76 M24-6g×70:22
442. Гайка ГОСТ 15524-70 M24:42
443. Шайба  ГОСТ 11371-78 25:22
444. Шпилька ГОСТ 22038-76 M24-6g×70:23
445. Гайка ГОСТ 15524-70 M24:43
446. Шайба  ГОСТ 11371-78 25:23
447. Шпилька ГОСТ 22038-76 M24-6g×70:24
448. Гайка ГОСТ 15524-70 M24:44
449. Шайба  ГОСТ 11371-78 25:24
450. Шпилька ГОСТ 22038-76 M24-6g×70:25
451. Гайка ГОСТ 15524-70 M24:45
452. Шайба  ГОСТ 11371-78 25:25
453. Шпилька ГОСТ 22038-76 M24-6g×70:26
454. Гайка ГОСТ 15524-70 M24:46
455. Шайба  ГОСТ 11371-78 25:26
456. Шпилька ГОСТ 22038-76 M24-6g×70:27
457. Гайка ГОСТ 15524-70 M24:47
458. Шайба  ГОСТ 11371-78 25:27
459. Шпилька ГОСТ 22038-76 M24-6g×70:28
460. Гайка ГОСТ 15524-70 M24:48
461. Шайба  ГОСТ 11371-78 25:28
462. Шпилька ГОСТ 22038-76 M24-6g×70:29
463. Гайка ГОСТ 15524-70 M24:49
464. Шайба  ГОСТ 11371-78 25:29
465. Шпилька ГОСТ 22038-76 M24-6g×70:30
466. Гайка ГОСТ 15524-70 M24:50
467. Шайба  ГОСТ 11371-78 25:30
468. Шпилька ГОСТ 22038-76 M24-6g×70:31
469. Гайка ГОСТ 15524-70 M24:51
470. Шайба  ГОСТ 11371-78 25:31
471. Шпилька ГОСТ 22038-76 M24-6g×70:32
472. Гайка ГОСТ 15524-70 M24:52
473. Шайба  ГОСТ 11371-78 25:32
474. Винт ГОСТ 11738-84 M 10x35:1 — Жесткий:129
475. Шайба  ГОСТ 11371-78 13:1 — Жесткий:128, Жесткий:129
476. Винт ГОСТ 11738-84 M 10x35:2
477. Шайба  ГОСТ 11371-78 13:5
478. Винт ГОСТ 11738-84 M 10x35:3
479. Шайба  ГОСТ 11371-78 13:6
480. Винт ГОСТ 11738-84 M 10x35:4
481. Шайба  ГОСТ 11371-78 13:7
482. Винт ГОСТ 11738-84 M 10x35:5
483. Шайба  ГОСТ 11371-78 13:8
484. Винт ГОСТ 11738-84 M 10x35:6
485. Шайба  ГОСТ 11371-78 13:9
486. Винт ГОСТ 11738-84 M 10x35:7
487. Шайба  ГОСТ 11371-78 13:10
488. Винт ГОСТ 11738-84 M 10x35:8
489. Шайба  ГОСТ 11371-78 13:11
490. Винт ГОСТ 11738-84 M 10x30:1 — Жесткий:131
491. Шайба  ГОСТ 11371-78 13:2 — Жесткий:130, Жесткий:131
492. Винт ГОСТ 11738-84 M 10x30:2
493. Шайба  ГОСТ 11371-78 13:12
494. Винт ГОСТ 11738-84 M 10x30:3
495. Шайба  ГОСТ 11371-78 13:13
496. Винт ГОСТ 11738-84 M 10x30:4
497. Шайба  ГОСТ 11371-78 13:14
498. Винт ГОСТ 11738-84 M 10x30:5
499. Шайба  ГОСТ 11371-78 13:15
500. Винт ГОСТ 11738-84 M 10x30:6
501. Шайба  ГОСТ 11371-78 13:16
502. Винт ГОСТ 11738-84 M 10x30:7
503. Шайба  ГОСТ 11371-78 13:17
504. Винт ГОСТ 11738-84 M 10x30:8
505. Шайба  ГОСТ 11371-78 13:18
506. Шайба  ГОСТ 11371-78 13:4 — Жесткий:134, Жесткий:135
507. Винт ГОСТ 11738-84 M 10x25:2 — Жесткий:135
508. Шайба  ГОСТ 11371-78 13:19
509. Винт ГОСТ 11738-84 M 10x25:3
510. Шайба  ГОСТ 11371-78 13:20
511. Винт ГОСТ 11738-84 M 10x25:4
512. Шайба  ГОСТ 11371-78 13:21
513. Винт ГОСТ 11738-84 M 10x25:5
514. Шайба  ГОСТ 11371-78 13:22
515. Винт ГОСТ 11738-84 M 10x25:6
516. Шайба  ГОСТ 11371-78 13:23
517. Винт ГОСТ 11738-84 M 10x25:7
518. Шайба  ГОСТ 11371-78 13:24
519. Винт ГОСТ 11738-84 M 10x25:8
520. Шайба  ГОСТ 11371-78 13:25
521. Винт ГОСТ 11738-84 M 10x25:9
522. Винт ГОСТ 11738-84 M 10x25:1 — Жесткий:133
523. Шайба  ГОСТ 11371-78 13:3 — Жесткий:133, Жесткий:132
524. Винт ГОСТ 11738-84 M 10x25:10
525. Шайба  ГОСТ 11371-78 13:26
526. Винт ГОСТ 11738-84 M 10x25:11
527. Шайба  ГОСТ 11371-78 13:27
528. Винт ГОСТ 11738-84 M 10x25:12
529. Шайба  ГОСТ 11371-78 13:28
530. Винт ГОСТ 11738-84 M 10x25:13
531. Шайба  ГОСТ 11371-78 13:29
532. Винт ГОСТ 11738-84 M 10x25:14
533. Шайба  ГОСТ 11371-78 13:30
534. Винт ГОСТ 11738-84 M 10x25:15
535. Шайба  ГОСТ 11371-78 13:31
536. Винт ГОСТ 11738-84 M 10x25:16
537. Шайба  ГОСТ 11371-78 13:32
538. Шпилька ГОСТ 22034-76 M20-6g×50:2 — Жесткий:122, Жесткий:124, Жесткий:123
539. Гайка ГОСТ 15521-70 M20:2 — Жесткий:124
540. Шайба ГОСТ 10450-78 19:2 — Жесткий:123
541. Шпилька ГОСТ 22034-76 M20-6g×50:14
542. Гайка ГОСТ 15521-70 M20:14
543. Шайба ГОСТ 10450-78 19:14
544. Шпилька ГОСТ 22034-76 M20-6g×50:15
545. Гайка ГОСТ 15521-70 M20:15
546. Шайба ГОСТ 10450-78 19:15
547. Шпилька ГОСТ 22034-76 M20-6g×50:16
548. Гайка ГОСТ 15521-70 M20:16
549. Шайба ГОСТ 10450-78 19:16
550. Шпилька ГОСТ 22034-76 M20-6g×50:17
551. Гайка ГОСТ 15521-70 M20:17
552. Шайба ГОСТ 10450-78 19:17
553. Шпилька ГОСТ 22034-76 M20-6g×50:18
554. Гайка ГОСТ 15521-70 M20:18
555. Шайба ГОСТ 10450-78 19:18
556. Шпилька ГОСТ 22034-76 M20-6g×50:19
557. Гайка ГОСТ 15521-70 M20:19
558. Шайба ГОСТ 10450-78 19:19
559. Шпилька ГОСТ 22034-76 M20-6g×50:20
560. Гайка ГОСТ 15521-70 M20:20
561. Шайба ГОСТ 10450-78 19:20
562. Шпилька ГОСТ 22034-76 M20-6g×50:21
563. Гайка ГОСТ 15521-70 M20:21
564. Шайба ГОСТ 10450-78 19:21
565. Шпилька ГОСТ 22034-76 M20-6g×50:22
566. Гайка ГОСТ 15521-70 M20:22
567. Шайба ГОСТ 10450-78 19:22
568. Гайка ГОСТ 15521-70 M20:3 — Жесткий:198
569. Шпилька ГОСТ 22034-76 M20-6g×50:3 — Жесткий:198, Жесткий:199
570. Шайба ГОСТ 10450-78 19:3 — Жесткий:199
571. Гайка ГОСТ 15521-70 M20:23
572. Шпилька ГОСТ 22034-76 M20-6g×50:23
573. Шайба ГОСТ 10450-78 19:23
574. Гайка ГОСТ 15521-70 M20:24
575. Шпилька ГОСТ 22034-76 M20-6g×50:24
576. Шайба ГОСТ 10450-78 19:24
577. Гайка ГОСТ 15521-70 M20:25
578. Шпилька ГОСТ 22034-76 M20-6g×50:25
579. Шайба ГОСТ 10450-78 19:25
580. Гайка ГОСТ 15521-70 M20:26
581. Шпилька ГОСТ 22034-76 M20-6g×50:26
582. Шайба ГОСТ 10450-78 19:26
583. Гайка ГОСТ 15521-70 M20:27
584. Шпилька ГОСТ 22034-76 M20-6g×50:27
585. Шайба ГОСТ 10450-78 19:27
586. Гайка ГОСТ 15521-70 M20:28
587. Шпилька ГОСТ 22034-76 M20-6g×50:28
588. Шайба ГОСТ 10450-78 19:28
589. Гайка ГОСТ 15521-70 M20:29
590. Шпилька ГОСТ 22034-76 M20-6g×50:29
591. Шайба ГОСТ 10450-78 19:29
592. Гайка ГОСТ 15521-70 M20:30
593. Шпилька ГОСТ 22034-76 M20-6g×50:30
594. Шайба ГОСТ 10450-78 19:30
595. Гайка ГОСТ 15521-70 M20:31
596. Шпилька ГОСТ 22034-76 M20-6g×50:31
597. Шайба ГОСТ 10450-78 19:31
598. Шпилька ГОСТ 22034-76 M20-6g×50:4 — Жесткий:200, Жесткий:201
599. Гайка ГОСТ 15521-70 M20:4 — Жесткий:200
600. Шайба ГОСТ 10450-78 19:4 — Жесткий:201
601. Шпилька ГОСТ 22034-76 M20-6g×50:32
602. Гайка ГОСТ 15521-70 M20:32
603. Шайба ГОСТ 10450-78 19:32
604. Шпилька ГОСТ 22034-76 M20-6g×50:33
605. Гайка ГОСТ 15521-70 M20:33
606. Шайба ГОСТ 10450-78 19:33
607. Шпилька ГОСТ 22034-76 M20-6g×50:34
608. Гайка ГОСТ 15521-70 M20:34
609. Шайба ГОСТ 10450-78 19:34
610. Шпилька ГОСТ 22034-76 M20-6g×50:35
611. Гайка ГОСТ 15521-70 M20:35
612. Шайба ГОСТ 10450-78 19:35
613. Шпилька ГОСТ 22034-76 M20-6g×50:36
614. Гайка ГОСТ 15521-70 M20:36
615. Шайба ГОСТ 10450-78 19:36
616. Шпилька ГОСТ 22034-76 M20-6g×50:37
617. Гайка ГОСТ 15521-70 M20:37
618. Шайба ГОСТ 10450-78 19:37
619. Шпилька ГОСТ 22034-76 M20-6g×50:38
620. Гайка ГОСТ 15521-70 M20:38
621. Шайба ГОСТ 10450-78 19:38
622. Шпилька ГОСТ 22034-76 M20-6g×50:39
623. Гайка ГОСТ 15521-70 M20:39
624. Шайба ГОСТ 10450-78 19:39
625. Шпилька ГОСТ 22034-76 M20-6g×50:40
626. Гайка ГОСТ 15521-70 M20:40
627. Шайба ГОСТ 10450-78 19:40
## Component patterns: (16 elements, first: Шпилька ГОСТ 22038-76 M20-6g×85:1 + Шайба ГОСТ 10450-78 21:1 + Гайка ГОСТ 15524-70 M20:1), (10 elements, first: Гайка ГОСТ 15521-70 M20:1 + Шпилька ГОСТ 22034-76 M20-6g×50:1 + Шайба ГОСТ 10450-78 19:1), (16 elements, first: Шпилька ГОСТ 22038-76 M24-6g×70:1 + Гайка ГОСТ 15524-70 M24:1 + Шайба  ГОСТ 11371-78 25:1), (8 elements, first: Винт ГОСТ 11738-84 M 10x35:1 + Шайба  ГОСТ 11371-78 13:1), (8 elements, first: Винт ГОСТ 11738-84 M 10x30:1 + Шайба  ГОСТ 11371-78 13:2), (8 elements, first: Шайба  ГОСТ 11371-78 13:4 + Винт ГОСТ 11738-84 M 10x25:2), (8 elements, first: Винт ГОСТ 11738-84 M 10x25:1 + Шайба  ГОСТ 11371-78 13:3), (10 elements, first: Шпилька ГОСТ 22034-76 M20-6g×50:2 + Гайка ГОСТ 15521-70 M20:2 + Шайба ГОСТ 10450-78 19:2), (10 elements, first: Гайка ГОСТ 15521-70 M20:3 + Шпилька ГОСТ 22034-76 M20-6g×50:3 + Шайба ГОСТ 10450-78 19:3), (10 elements, first: Шпилька ГОСТ 22034-76 M20-6g×50:4 + Гайка ГОСТ 15521-70 M20:4 + Шайба ГОСТ 10450-78 19:4)
## Relationships (305: WeldJoint 283, Flush 10, RevoluteJoint 8, Mate 2, CylindricalJoint 2)
- Совмещение:1 [Mate] (115 mm): Верхняя часть поршня_CPY:1 ↔ Крышка цилиндра 1_CPY:1
- Заподлицо:1 [Flush] (449.5 mm): Шайба  ГОСТ 11371-78 25:1
- Совмещение:2 [Mate] (449.5 mm): Шайба  ГОСТ 11371-78 25:2
- Заподлицо:2 [Flush] (-412.5 mm): Цилиндр2_CPY:1
- Заподлицо:5 [Flush]: Фонарь_CPY:1 ↔ Прокладка крышки фонаря 1_CPY:1
- Заподлицо:4 [Flush]: Фонарь_CPY:1 ↔ Прокладка крышки фонаря 1_CPY:1
- Заподлицо:7 [Flush]: Фонарь_CPY:1 ↔ Прокладка крышки фонаря 2_CPY:1
- Заподлицо:6 [Flush]: Фонарь_CPY:1 ↔ Прокладка крышки фонаря 2_CPY:1
- Цилиндрический:2 [CylindricalJoint]: Фонарь_CPY:1 ↔ Башмак_CPY:1
- Жесткий:4 [WeldJoint]: Башмак_CPY:1 ↔ Крейцкопф_CPY:1